# Autodesk Inventor assembly: 1510-2898-A-0700
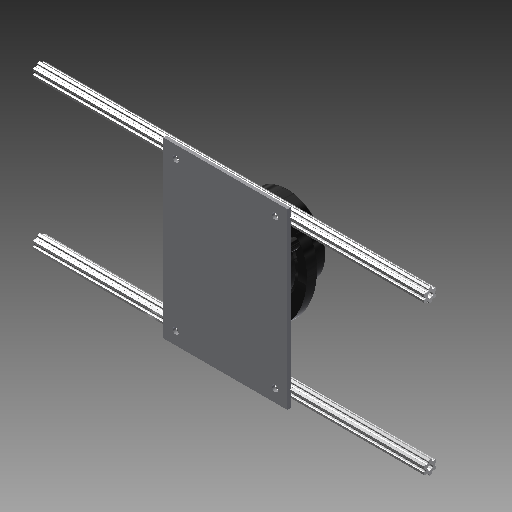
[picture p0: Inventor's stored thumbnail of the model, 512x512]
Saved by Autodesk Inventor 2017 (Build 210142000, 142)
## iProperties
Created: 2016-10-09
Part Number: 1510-2898-A-0700
Document SubType Name: Assembly
Designer: gus
Mass: 529.499 g
Surface Area: 1690.81 cm^2
Volume: 394.779 cm^3
Density: 1.34125 g/cm^3
Author: gus
## Documents named in this file (4)
- \\Mac\Home\Desktop\bunnybots 2016\15102898-16-Bunnybot-CAD\Bunnybot-Night_Fury\15102898-16-A-0000\15102898-16-A-0700\1510-2898-A-0700.iam
- \\Mac\Home\Desktop\bunnybots 2016\15102898-16-Bunnybot-CAD\Bunnybot-Night_Fury\15102898-16-A-0000\15102898-16-A-0700\xv11LidarAssy.ipt
- \\Mac\Home\Desktop\bunnybots 2016\15102898-16-Bunnybot-CAD\Bunnybot-Night_Fury\15102898-16-A-0000\15102898-16-A-0700\Imported Components\Churro 15750.ipt
- \\Mac\Home\Desktop\bunnybots 2016\15102898-16-Bunnybot-CAD\Bunnybot-Night_Fury\15102898-16-A-0000\15102898-16-A-0700\1512898-16-P-0701.ipt
## Components (4 placed, 3 different names)
1. xv11LidarAssy:1 — Flush:1, Mate:8, Mate:9
2. Churro 15750:1 — Mate:2, Mate:3, Mate:4
3. 1512898-16-P-0701:1 — Mate:2, Mate:3, Mate:4, Mate:5, Mate:6, Mate:7, Flush:1, Mate:8, Mate:9
4. Churro 15750:2 — Mate:5, Mate:6, Mate:7
## Relationships (9: Mate 8, Flush 1)
- Mate:2: Churro 15750:1 ↔ 1512898-16-P-0701:1
- Mate:3: Churro 15750:1 ↔ 1512898-16-P-0701:1
- Mate:4: Churro 15750:1 ↔ 1512898-16-P-0701:1
- Mate:5: 1512898-16-P-0701:1 ↔ Churro 15750:2
- Mate:6: 1512898-16-P-0701:1 ↔ Churro 15750:2
- Mate:7: 1512898-16-P-0701:1 ↔ Churro 15750:2
- Flush:1 (28.575 mm): xv11LidarAssy:1 ↔ 1512898-16-P-0701:1
- Mate:8: xv11LidarAssy:1 ↔ 1512898-16-P-0701:1
- Mate:9 (-11.1125 mm): xv11LidarAssy:1 ↔ 1512898-16-P-0701:1
